# Autodesk Inventor assembly: RSL light mount
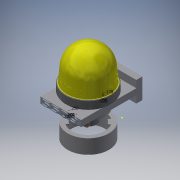
[picture p0: Inventor's stored thumbnail of the model, 180x180]
Saved by Autodesk Inventor 2019 (Build 230136000, 136)
## iProperties
Created: 2019-02-11
Part Number: RSL light mount
Document SubType Name: Assembly
Designer: josh
Author: josh
## Documents named in this file (4)
- D:\Synthesis Robots\Epsilon\RSL light mount.iam
- D:\Synthesis Robots\Epsilon\Epsilon elavator lift\RSL mount.ipt
- D:\Synthesis Robots\Epsilon\Epsilon elavator lift\am-3583 Generic RSL.ipt
- D:\Synthesis Robots\Epsilon\Epsilon elavator lift\RSL light mount (guard 1).ipt
## Components (3 placed, 3 different names)
1. RSL mount:1 — Mate:1, Mate:2, Mate:3
2. am-3583 Generic RSL:1 — Mate:1, Mate:2
3. RSL light mount (guard 1):1 — Mate:3
## Relationships (3: Mate 3)
- Mate:1: RSL mount:1 ↔ am-3583 Generic RSL:1
- Mate:2: RSL mount:1 ↔ am-3583 Generic RSL:1
- Mate:3: RSL mount:1 ↔ RSL light mount (guard 1):1
